# Autodesk Inventor assembly: Final submission assembly
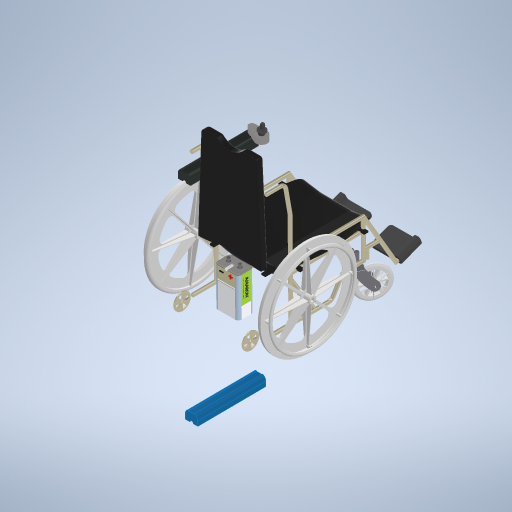
[picture p0: Inventor's stored thumbnail of the model, 512x512]
Saved by Autodesk Inventor 2023 (Build 270158000, 158)
## iProperties
Created: 2023-11-16
Part Number: Final submission assembly
Document SubType Name: Assembly
Designer: Raghav
Author: Raghav
## Documents named in this file (16)
- C:\Users\Public\Documents\Autodesk\Inventor 2023\EG Project\EG FINAL\assembly.iam parts\Final submission assembly.iam
- C:\Users\Vivek Rajput\Documents\EG\Workspaces\Workspace\EG Project - Copy\Side frame.ipt
- C:\Users\Vivek Rajput\Documents\EG\Workspaces\Workspace\EG Project - Copy\Rear wheel.ipt
- C:\Users\Dell\OneDrive - iitgn.ac.in\Sem_1\ES-101\Course Project\Final assembly\Motor.ipt
- C:\Users\Public\Documents\Autodesk\Inventor 2023\EG Project\EG FINAL\assembly.iam parts\battery eg 26.ipt
- C:\Users\Public\Documents\Autodesk\Inventor 2023\EG Project\EG FINAL\assembly.iam parts\Rahul_Foot rest.ipt
- C:\Users\Vivek Rajput\Documents\EG\Workspaces\Workspace\Castorfork.ipt
- C:\Users\Vivek Rajput\Documents\EG\Workspaces\Workspace\EG Project - Copy\zfront wheel.ipt
- C:\Users\Public\Documents\Autodesk\Inventor 2023\EG Project\EG FINAL\assembly.iam parts\Raghav_Anti Tip.ipt
- C:\Users\Vivek Rajput\Documents\EG\Workspaces\Workspace\EG Project - Copy\arm rest final 1.ipt
- C:\Users\Public\Documents\Autodesk\Inventor 2023\EG Project\EG FINAL\assembly.iam parts\G26_P999999[4].ipt
- C:\Users\Public\Documents\Autodesk\Inventor 2023\EG Project\EG FINAL\assembly.iam parts\G26_P999999[4L].ipt
- C:\Users\Public\Documents\Autodesk\Inventor 2023\EG Project\EG FINAL\assembly.iam parts\Rachit_Seat.ipt
- C:\Users\Public\Documents\Autodesk\Inventor 2023\EG Project\EG FINAL\assembly.iam parts\Rahul_Backrest.ipt
- C:\Users\Public\Documents\Autodesk\Inventor 2023\EG Project\EG FINAL\assembly.iam parts\Joystick base.ipt
- C:\Users\Public\Documents\Autodesk\Inventor 2023\EG Project\EG FINAL\assembly.iam parts\Joystick upper.ipt
## Components (22 placed, 15 different names)
1. Side frame:1 — Rotational:1, Rotational:2, Rotational:3, Rotational:4, Rigid:1, Rotational:5, Rotational:6, Mate:1, Mate:2, Rotational:11, Rotational:12, Rigid:2, Rigid:3, Mate:3, Rigid:4, Mate:4, Rigid:5, Rigid:6
2. Rear wheel:1 — Rotational:5, Rotational:7
3. Rear wheel:2 — Rotational:6, Rotational:8
4. Motor:1 — Rotational:7, Mate:1
5. Motor:2 — Rotational:8, Mate:2
6. battery eg 26:1 — Rigid:1
7. Rahul_Foot rest:1 — Rotational:11
8. Rahul_Foot rest:2 — Rotational:12
9. Castorfork:1 — Rotational:3, Rotational:9
10. Castorfork:2 — Rotational:4, Rotational:10
11. zfront wheel:1 — Rotational:10
12. zfront wheel:2 — Rotational:9
13. Raghav_Anti Tip:1 — Rotational:2
14. Raghav_Anti Tip:2 — Rotational:1
15. arm rest final 1:1 — Rigid:2, Rigid:8
16. arm rest final 1:2 — Rigid:3
17. G26_P999999[4]:1 — Mate:4, Rigid:5
18. G26_P999999[4L]:1 — Mate:3, Rigid:4
19. Rachit_Seat:1 — Rigid:6, Rigid:7
20. Rahul_Backrest:1 — Rigid:7
21. Joystick base:1 — Rigid:8, Ball:1
22. Joystick upper:1 — Ball:1
## Relationships (25: RevoluteJoint 12, WeldJoint 8, Mate 4, BallJoint 1)
- Rotational:1 [RevoluteJoint]: Side frame:1 ↔ Raghav_Anti Tip:2
- Rotational:2 [RevoluteJoint]: Side frame:1 ↔ Raghav_Anti Tip:1
- Rotational:3 [RevoluteJoint]: Side frame:1 ↔ Castorfork:1
- Rotational:4 [RevoluteJoint]: Side frame:1 ↔ Castorfork:2
- Rigid:1 [WeldJoint]: Side frame:1 ↔ battery eg 26:1
- Rotational:5 [RevoluteJoint]: Side frame:1 ↔ Rear wheel:1
- Rotational:6 [RevoluteJoint]: Side frame:1 ↔ Rear wheel:2
- Rotational:7 [RevoluteJoint]: Rear wheel:1 ↔ Motor:1
- Mate:1: Side frame:1 ↔ Motor:1
- Rotational:8 [RevoluteJoint]: Rear wheel:2 ↔ Motor:2
- Mate:2: Side frame:1 ↔ Motor:2
- Rotational:9 [RevoluteJoint]: Castorfork:1 ↔ zfront wheel:2
- Rotational:10 [RevoluteJoint]: Castorfork:2 ↔ zfront wheel:1
- Rotational:11 [RevoluteJoint]: Side frame:1 ↔ Rahul_Foot rest:1
- Rotational:12 [RevoluteJoint]: Side frame:1 ↔ Rahul_Foot rest:2
- Rigid:2 [WeldJoint]: Side frame:1 ↔ arm rest final 1:1
- Rigid:3 [WeldJoint]: Side frame:1 ↔ arm rest final 1:2
- Mate:3: Side frame:1 ↔ G26_P999999[4L]:1
- Rigid:4 [WeldJoint]: Side frame:1 ↔ G26_P999999[4L]:1
- Mate:4: Side frame:1 ↔ G26_P999999[4]:1
- Rigid:5 [WeldJoint]: Side frame:1 ↔ G26_P999999[4]:1
- Rigid:6 [WeldJoint]: Side frame:1 ↔ Rachit_Seat:1
- Rigid:7 [WeldJoint]: Rachit_Seat:1 ↔ Rahul_Backrest:1
- Rigid:8 [WeldJoint]: arm rest final 1:1 ↔ Joystick base:1
- Ball:1: Joystick base:1 ↔ Joystick upper:1
